# Autodesk Inventor assembly: Framing_For_First_Floor_Back_Window
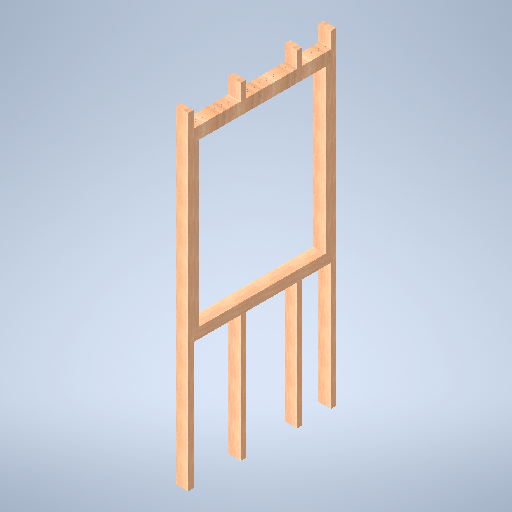
[picture p0: Inventor's stored thumbnail of the model, 512x512]
Saved by Autodesk Inventor 2025.1 (Build 291241020, 241B)
## iProperties
Created: 2024-09-15
Part Number: Framing_For_First_Floor_Back_Window
Document SubType Name: Assembly
Designer: Tom
Author: Tom
## Documents named in this file (7)
- C:\Users\Tom\Documents\Inventor\Mobility\Additional_Building\Framing_For_Back_Living_Room_Window.iam
- C:\Users\Tom\Documents\Inventor\Mobility\Additional_Building\Stud_With_Height_93_Inches.ipt
- C:\Users\Tom\Documents\Inventor\Mobility\Additional_Building\Sill_Plate_With_Length_39_Inches.ipt
- C:\Users\Tom\Documents\Inventor\Mobility\Additional_Building\Stud_With_Height_46_Inches.ipt
- C:\Users\Tom\Documents\Inventor\Mobility\Additional_Building\Header_With_Dimensions_3.5_x_3.5_x_39_Inches.iam
- C:\Users\Tom\Documents\Inventor\Mobility\Additional_Building\Stud_With_Height_4.5625_Inches.ipt
- C:\Users\Tom\Documents\Inventor\Mobility\Additional_Building\Stud_With_Height_35.9375_Inches.ipt
## Components (11 placed, 6 different names)
1. Stud_With_Height_93_Inches:59 — Mate:46, Flush:48, Mate:48, Mate:50, Mate:57, Flush:58, Flush:59
2. Sill_Plate_With_Length_39_Inches:1 — Mate:46, Flush:48, Mate:47, Flush:49, Mate:55
3. Sill_Plate_With_Length_39_Inches:2 — Mate:47, Mate:48, Flush:49, Mate:49, Flush:50, Mate:53, Flush:52, Flush:53
4. Stud_With_Height_46_Inches:1 — Mate:49, Mate:50, Flush:50, Mate:56, Flush:56
5. Stud_With_Height_46_Inches:2 — Mate:53, Flush:52, Flush:53
6. Stud_With_Height_93_Inches:61 — Mate:55
7. Header_With_Dimensions_3.5_x_3.5_x_39_Inches:1 [sub-assembly] — Mate:56, Mate:57, Flush:56, Mate:59, Flush:57
8. Stud_With_Height_4.5625_Inches:1 — Mate:59, Flush:57, Flush:58
9. Stud_With_Height_4.5625_Inches:2
10. Stud_With_Height_35.9375_Inches:1 — Flush:59
11. Stud_With_Height_35.9375_Inches:2
## Component patterns: (2 elements, first: Stud_With_Height_4.5625_Inches:1), (2 elements, first: Stud_With_Height_35.9375_Inches:1)
## Relationships (19: Mate 10, Flush 9)
- Mate:46: Stud_With_Height_93_Inches:59 ↔ Sill_Plate_With_Length_39_Inches:1
- Flush:48: Stud_With_Height_93_Inches:59 ↔ Sill_Plate_With_Length_39_Inches:1
- Mate:47: Sill_Plate_With_Length_39_Inches:1 ↔ Sill_Plate_With_Length_39_Inches:2
- Mate:48: Stud_With_Height_93_Inches:59 ↔ Sill_Plate_With_Length_39_Inches:2
- Flush:49: Sill_Plate_With_Length_39_Inches:1 ↔ Sill_Plate_With_Length_39_Inches:2
- Mate:49: Sill_Plate_With_Length_39_Inches:2 ↔ Stud_With_Height_46_Inches:1
- Mate:50: Stud_With_Height_93_Inches:59 ↔ Stud_With_Height_46_Inches:1
- Flush:50: Sill_Plate_With_Length_39_Inches:2 ↔ Stud_With_Height_46_Inches:1
- Mate:53: Sill_Plate_With_Length_39_Inches:2 ↔ Stud_With_Height_46_Inches:2
- Flush:52: Sill_Plate_With_Length_39_Inches:2 ↔ Stud_With_Height_46_Inches:2
- Flush:53: Sill_Plate_With_Length_39_Inches:2 ↔ Stud_With_Height_46_Inches:2
- Mate:55: Sill_Plate_With_Length_39_Inches:1 ↔ Stud_With_Height_93_Inches:61
- Mate:56: Stud_With_Height_46_Inches:1 ↔ Header_With_Dimensions_3.5_x_3.5_x_39_Inches:1
- Mate:57: Stud_With_Height_93_Inches:59 ↔ Header_With_Dimensions_3.5_x_3.5_x_39_Inches:1
- Flush:56: Stud_With_Height_46_Inches:1 ↔ Header_With_Dimensions_3.5_x_3.5_x_39_Inches:1
- Mate:59: Header_With_Dimensions_3.5_x_3.5_x_39_Inches:1 ↔ Stud_With_Height_4.5625_Inches:1
- Flush:57: Header_With_Dimensions_3.5_x_3.5_x_39_Inches:1 ↔ Stud_With_Height_4.5625_Inches:1
- Flush:58 (379.4125 mm): Stud_With_Height_93_Inches:59 ↔ Stud_With_Height_4.5625_Inches:1
- Flush:59 (379.4125 mm): Stud_With_Height_93_Inches:59 ↔ Stud_With_Height_35.9375_Inches:1
